# Autodesk Inventor assembly: RPi Desk Case Assem
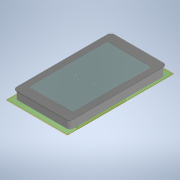
[picture p0: Inventor's stored thumbnail of the model, 180x180]
Saved by Autodesk Inventor 2021 (Build 250183000, 183)
## iProperties
Created: 2022-06-16
Part Number: RPi Desk Case Assem
Document SubType Name: Assembly
Designer: cmzgt
Author: cmzgt
## Documents named in this file (5)
- D:\Projects\3D Designs\RPi Desk Case\RPi Desk Case Assem.iam
- D:\Projects\3D Designs\RPi Desk Case\References\Rpi_Touchscreen_7in_Logo.ipt
- D:\Projects\3D Designs\RPi Desk Case\RPi Desk Case.ipt
- D:\Projects\3D Designs\RPi Desk Case\References\Raspberry Pi 3.ipt
- D:\Projects\3D Designs\RPi Desk Case\RPi Case.ipt
## Components (4 placed, 4 different names)
1. Rpi_Touchscreen_7in_Logo:1 — Flush:1, Flush:4, Mate:1, Mate:2, Angle:1, Mate:3
2. RPi Desk Case:1 — Flush:1, Flush:4, Flush:5, Flush:6, Flush:7
3. Raspberry Pi 3:1 — Mate:1, Mate:2, Angle:1, Mate:3
4. RPi Case:1 — Flush:5, Flush:6, Flush:7
## Relationships (9: Flush 5, Mate 3, Angle 1)
- Flush:1: Rpi_Touchscreen_7in_Logo:1 ↔ RPi Desk Case:1
- Flush:4 (15.621 mm): Rpi_Touchscreen_7in_Logo:1 ↔ RPi Desk Case:1
- Mate:1: Rpi_Touchscreen_7in_Logo:1 ↔ Raspberry Pi 3:1
- Mate:2: Rpi_Touchscreen_7in_Logo:1 ↔ Raspberry Pi 3:1
- Angle:1 (0 deg): Rpi_Touchscreen_7in_Logo:1 ↔ Raspberry Pi 3:1
- Mate:3 (12.7 mm): Rpi_Touchscreen_7in_Logo:1 ↔ Raspberry Pi 3:1
- Flush:5: RPi Desk Case:1 ↔ RPi Case:1
- Flush:6: RPi Desk Case:1 ↔ RPi Case:1
- Flush:7: RPi Desk Case:1 ↔ RPi Case:1
